# Autodesk Inventor assembly: Sliced Unit
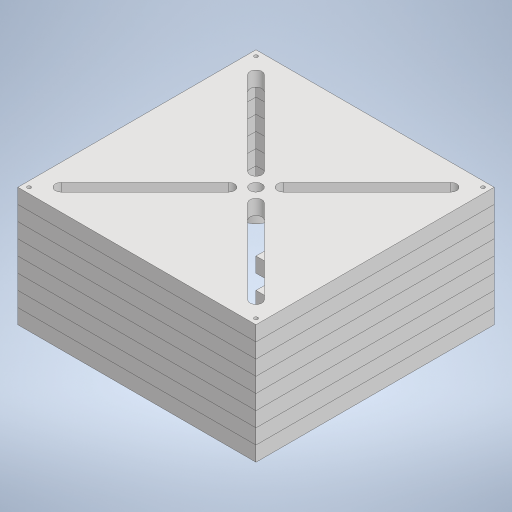
[picture p0: Inventor's stored thumbnail of the model, 512x512]
Saved by Autodesk Inventor 2023 (Build 270158000, 158)
## iProperties
Created: 2023-04-21
Part Number: Sliced Unit
Document SubType Name: Assembly
Designer: byrne
Author: byrne
## Documents named in this file (6)
- C:\Users\byrne\OneDrive\Documents\Inventor\RAI\Sliced Unit.iam
- C:\Users\byrne\OneDrive\Documents\Inventor\RAI\Layer 1.ipt
- C:\Users\byrne\OneDrive\Documents\Inventor\RAI\Layer 2.ipt
- C:\Users\byrne\OneDrive\Documents\Inventor\RAI\Layer 3.ipt
- C:\Users\byrne\OneDrive\Documents\Inventor\RAI\Layer 4.ipt
- C:\Users\byrne\OneDrive\Documents\Inventor\RAI\Layer 5.ipt
## Components (8 placed, 5 different names)
1. Layer 1:1 — Insert:1, Insert:2
2. Layer 2:1 — Insert:1, Insert:2, Insert:3, Insert:4
3. Layer 3:1 — Insert:3, Insert:4, Insert:5, Insert:6
4. Layer 4:1 — Insert:5, Insert:6, Insert:11, Insert:12
5. Layer 4:2 — Insert:8, Insert:10, Insert:11, Insert:12
6. Layer 4:3 — Insert:7, Insert:8, Insert:9, Insert:10
7. Layer 4:4 — Insert:7, Insert:9, Insert:13, Insert:14
8. Layer 5:1 — Insert:13, Insert:14
## Relationships (14: Insert 14)
- Insert:1: Layer 1:1 ↔ Layer 2:1
- Insert:2: Layer 1:1 ↔ Layer 2:1
- Insert:3: Layer 2:1 ↔ Layer 3:1
- Insert:4: Layer 2:1 ↔ Layer 3:1
- Insert:5: Layer 3:1 ↔ Layer 4:1
- Insert:6: Layer 3:1 ↔ Layer 4:1
- Insert:7: Layer 4:3 ↔ Layer 4:4
- Insert:8: Layer 4:2 ↔ Layer 4:3
- Insert:9: Layer 4:3 ↔ Layer 4:4
- Insert:10: Layer 4:2 ↔ Layer 4:3
- Insert:11: Layer 4:1 ↔ Layer 4:2
- Insert:12: Layer 4:1 ↔ Layer 4:2
- Insert:13: Layer 4:4 ↔ Layer 5:1
- Insert:14: Layer 4:4 ↔ Layer 5:1
